# Autodesk Inventor assembly: y_plate_assembly_left
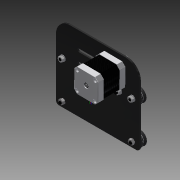
[picture p0: Inventor's stored thumbnail of the model, 180x180]
Saved by Autodesk Inventor 2014 (Build 180170000, 170)
## iProperties
Created: 2013-07-17
Part Number: y_plate_assembly_left
Document SubType Name: Assembly
Designer: Edward
Author: Edward
## Documents named in this file (14)
- C:\Users\Edward\Desktop\Shapeoko_v2.0\shapeoko_lowpro\y_plate_assembly_left.iam
- C:\Users\Edward\Desktop\Shapeoko_v2.0\motor_mount_v2_MIR.ipt
- C:\Users\Edward\Desktop\Shapeoko_v2.0\B18033_MIR.ipt
- C:\Users\Edward\Desktop\Shapeoko_v2.0\B30037_MIR.iam
- C:\Users\Edward\Desktop\Shapeoko_v2.0\SM-H03_MIR.ipt
- C:\Users\Edward\Desktop\Shapeoko_v2.0\91239A233_MIR.ipt
- C:\Users\Edward\Desktop\Shapeoko_v2.0\SM-H04_MIR.ipt
- C:\Users\Edward\Downloads\M1173041- NEMA 17_MIR.ipt
- C:\Users\Edward\Desktop\Shapeoko_v2.0\B30041_MIR.iam
- C:\Users\Edward\Desktop\Shapeoko_v2.0\91239A236_MIR.ipt
- C:\Users\Edward\Desktop\Shapeoko_v2.0\AS38-12-20_MIR.ipt
- C:\Users\Edward\Desktop\Shapeoko_v2.0\a_6a51-020df0606_MIR.ipt
- C:\Users\Edward\Desktop\Shapeoko_v2.0\91290A113.ipt
- C:\Users\Edward\Desktop\Shapeoko_v2.0\91166A210.ipt
## Components (41 placed, 13 different names)
1. motor_mount_v2_MIR:1 — Insert:10, Insert:11, Mate:3, Insert:12, Insert:18, Insert:20, Mate:5, Insert:19, Insert:21, Insert:25, Insert:27, Insert:28, Insert:29, Insert:30, Insert:31
2. B18033_MIR:1 — Insert:10, Mate:2
3. B30037_MIR:1 [sub-assembly] — Insert:5, Insert:6
4. SM-H03_MIR:1 — Insert:11, Insert:5
5. 91239A233_MIR:1 — Insert:6
6. SM-H04_MIR:1 — Insert:7
7. SM-H03_MIR:2 — Mate:3, Insert:8
8. SM-H03_MIR:3 — Insert:12, Insert:7
9. 91239A233_MIR:2 — Mate:2, Insert:9
10. B30037_MIR:2 [sub-assembly] — Insert:9, Insert:8
11. B18033_MIR:2 — Insert:18, Mate:4
12. B30037_MIR:3 [sub-assembly] — Insert:13, Insert:14
13. SM-H03_MIR:4 — Insert:20, Insert:13
14. 91239A233_MIR:3 — Insert:14
15. SM-H04_MIR:2 — Insert:15
16. SM-H03_MIR:5 — Mate:5, Insert:16
17. SM-H03_MIR:6 — Insert:19, Insert:15
18. 91239A233_MIR:4 — Mate:4, Insert:17
19. B30037_MIR:4 [sub-assembly] — Insert:17, Insert:16
20. M1173041- NEMA 17_MIR:1 — Insert:21, Mate:6
21. a_6a51-020df0606_MIR:1 — Mate:6
22. 91290A113:1
23. 91166A210:1 — Insert:30
24. 91290A113:2
25. 91166A210:2 — Insert:31
26. 91290A113:3
27. 91166A210:3 — Insert:29
28. 91290A113:4
29. 91166A210:4 — Insert:28
30. 91239A236_MIR:1 — Insert:22
31. B30041_MIR:1 [sub-assembly] — Insert:22, Insert:23
32. AS38-12-20_MIR:1 — Insert:23, Insert:24
33. SM-H03_MIR:7 — Insert:25, Insert:24
34. SM-H03_MIR:8 — Insert:27, Insert:26
35. SM-H04_MIR:4 — Insert:26
36. 91239A236_MIR:2
37. B30041_MIR:2 [sub-assembly]
38. AS38-12-20_MIR:2
39. SM-H03_MIR:9
40. SM-H03_MIR:10
41. SM-H04_MIR:5
## Component patterns: (2 elements, first: 91239A236_MIR:1 + B30041_MIR:1 + AS38-12-20_MIR:1 + SM-H03_MIR:7 + SM-H03_MIR:8 + SM-H04_MIR:4)
## Relationships (36: Insert 31, Mate 5)
- Insert:10: motor_mount_v2_MIR:1 ↔ B18033_MIR:1
- Insert:11: motor_mount_v2_MIR:1 ↔ SM-H03_MIR:1
- Insert:5: B30037_MIR:1 ↔ SM-H03_MIR:1
- Insert:6: B30037_MIR:1 ↔ 91239A233_MIR:1
- Mate:3: motor_mount_v2_MIR:1 ↔ SM-H03_MIR:2
- Insert:12: motor_mount_v2_MIR:1 ↔ SM-H03_MIR:3
- Insert:7: SM-H04_MIR:1 ↔ SM-H03_MIR:3
- Mate:2: B18033_MIR:1 ↔ 91239A233_MIR:2
- Insert:9: 91239A233_MIR:2 ↔ B30037_MIR:2
- Insert:8: SM-H03_MIR:2 ↔ B30037_MIR:2
- Insert:18: motor_mount_v2_MIR:1 ↔ B18033_MIR:2
- Insert:20: motor_mount_v2_MIR:1 ↔ SM-H03_MIR:4
- Insert:13: B30037_MIR:3 ↔ SM-H03_MIR:4
- Insert:14: B30037_MIR:3 ↔ 91239A233_MIR:3
- Mate:5: motor_mount_v2_MIR:1 ↔ SM-H03_MIR:5
- Insert:19: motor_mount_v2_MIR:1 ↔ SM-H03_MIR:6
- Insert:15: SM-H04_MIR:2 ↔ SM-H03_MIR:6
- Mate:4: B18033_MIR:2 ↔ 91239A233_MIR:4
- Insert:17: 91239A233_MIR:4 ↔ B30037_MIR:4
- Insert:16: SM-H03_MIR:5 ↔ B30037_MIR:4
- Insert:21: motor_mount_v2_MIR:1 ↔ M1173041- NEMA 17_MIR:1
- Insert:22: 91239A236_MIR:1 ↔ B30041_MIR:1
- Insert:23: B30041_MIR:1 ↔ AS38-12-20_MIR:1
- Insert:25: motor_mount_v2_MIR:1 ↔ SM-H03_MIR:7
- Insert:24: AS38-12-20_MIR:1 ↔ SM-H03_MIR:7
- Mate:6: M1173041- NEMA 17_MIR:1 ↔ a_6a51-020df0606_MIR:1
- Insert:27: motor_mount_v2_MIR:1 ↔ SM-H03_MIR:8
- Insert:26: SM-H03_MIR:8 ↔ SM-H04_MIR:4
- [Insert]: 91290A113:1 ↔ 91166A210:1
- [Insert]: 91290A113:2 ↔ 91166A210:2
- [Insert]: 91290A113:3 ↔ 91166A210:3
- [Insert]: 91290A113:4 ↔ 91166A210:4
- Insert:28: motor_mount_v2_MIR:1 ↔ 91166A210:4
- Insert:29: motor_mount_v2_MIR:1 ↔ 91166A210:3
- Insert:30: motor_mount_v2_MIR:1 ↔ 91166A210:1
- Insert:31: motor_mount_v2_MIR:1 ↔ 91166A210:2
## Named parameters: d182_d39 = 0 mm, d35_d182_d39 = 0 mm, d36_d182_d39 = 0 mm, d37_d182_d39 = 0 mm
